# Autodesk Inventor assembly: 60-J6
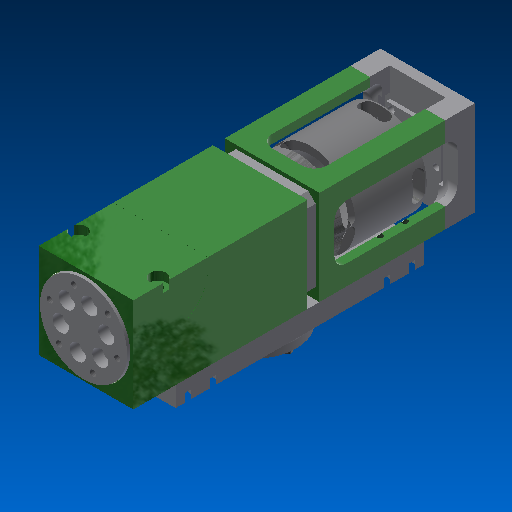
[picture p0: Inventor's stored thumbnail of the model, 512x512]
Saved by Autodesk Inventor 2018 (Build 220112000, 112)
## iProperties
Created: 2020-07-02
Part Number: 60-J6
Document SubType Name: Assembly
Designer: Bunny320
Author: Bunny320
## Documents named in this file (11)
- D:\Seerosenstr\sechs\4-CAD\60-J6.iam
- D:\Seerosenstr\sechs\4-CAD\motor unit 2820.iam
- D:\Seerosenstr\sechs\4-CAD\standardParts\61705-2RZ\W 61705-2RZ.iam
- D:\Seerosenstr\sechs\4-CAD\standardParts\Pololu mounting hub\pololu-universal-aluminum-mounting-hub-for-6mm-shaft-m3-holes.ipt
- C:\Users\Bunny320\Documents\Inventor\Content Center Files\R2018\en-US\ISO 10642(2)\ISO 10642  - M3  x  12.ipt
- C:\Users\mo\Documents\Inventor\Content Center Files\R2018\en-US\ISO 4762(1)\DIN EN ISO 4762 - M3 x 12.ipt
- C:\Users\Bunny320\Documents\Inventor\Content Center Files\R2018\en-US\ISO 4762(1)\DIN EN ISO 4762 - M3 x 8.ipt
- D:\Seerosenstr\sechs\4-CAD\602-gearbox-housing.ipt
- D:\Seerosenstr\sechs\4-CAD\601-flange.ipt
- D:\Seerosenstr\sechs\4-CAD\602-gearbox-housing-cap.ipt
- D:\Seerosenstr\sechs\4-CAD\605-output disk.ipt
## Components (25 placed, 10 different names)
1. motor unit 2820:1 [sub-assembly] — Flush:1, Flush:2, Flush:3, Mate:1, Mate:2, Mate:3, Mate:69, Mate:70
2. 602-gearbox-housing:1 — Mate:1, Mate:2, Mate:3, Mate:6, Mate:15, Mate:16, Mate:17, Mate:18, Mate:19, Mate:20, Mate:21, Mate:22, Mate:74, Mate:76, Mate:77
3. W 61705-2RZ:1 [sub-assembly] — Mate:6, Mate:71, Mate:73, Mate:74, Mate:75
4. pololu-universal-aluminum-mounting-hub-for-6mm-shaft-m3-holes:1 — Mate:72, Mate:73
5. 601-flange:1 — Mate:15, Mate:27, Mate:28, Mate:29, Mate:30, Mate:31, Mate:32, Mate:33, Mate:34, Mate:35, Mate:36, Mate:37, Mate:38, Mate:39, Mate:40, Mate:41, Mate:42, Mate:43, Mate:44, Mate:45, Mate:46, Mate:47, Mate:48, Mate:49, Mate:50, Mate:51, Mate:52, Mate:53, Mate:54, Mate:69, Mate:70
6. 602-gearbox-housing-cap:1 — Mate:16, Mate:17, Mate:18, Mate:76, Mate:77
7. 605-output disk:1 — Mate:71, Mate:72, Mate:75
8. DIN EN ISO 10642 M3  x  12:1 — Mate:19
9. DIN EN ISO 10642 M3  x  12:2 — Mate:20
10. DIN EN ISO 10642 M3  x  12:3 — Mate:21
11. DIN EN ISO 10642 M3  x  12:4 — Mate:22
12. DIN EN ISO 4762 M3 x 12:1 — Mate:27, Mate:28
13. DIN EN ISO 4762 M3 x 12:2 — Mate:29, Mate:30
14. DIN EN ISO 4762 M3 x 12:3 — Mate:31, Mate:32
15. DIN EN ISO 4762 M3 x 12:4 — Mate:33, Mate:34
16. DIN EN ISO 4762 M3 x 12:5 — Mate:35, Mate:36
17. DIN EN ISO 4762 M3 x 12:6 — Mate:37, Mate:38
18. DIN EN ISO 4762 M3 x 8:1 — Mate:39, Mate:40
19. DIN EN ISO 4762 M3 x 8:2 — Mate:41, Mate:42
20. DIN EN ISO 4762 M3 x 8:3 — Mate:43, Mate:44
21. DIN EN ISO 4762 M3 x 8:4 — Mate:45, Mate:46
22. DIN EN ISO 4762 M3 x 8:5 — Mate:47, Mate:48
23. DIN EN ISO 4762 M3 x 8:6 — Mate:49, Mate:50
24. DIN EN ISO 4762 M3 x 8:7 — Mate:51, Mate:52
25. DIN EN ISO 4762 M3 x 8:8 — Mate:53, Mate:54
## Relationships (52: Mate 49, Flush 3)
- Flush:1: motor unit 2820:1
- Flush:2: motor unit 2820:1
- Flush:3: motor unit 2820:1
- Mate:1: motor unit 2820:1 ↔ 602-gearbox-housing:1
- Mate:2: motor unit 2820:1 ↔ 602-gearbox-housing:1
- Mate:3: motor unit 2820:1 ↔ 602-gearbox-housing:1
- Mate:6: 602-gearbox-housing:1 ↔ W 61705-2RZ:1
- Mate:15: 602-gearbox-housing:1 ↔ 601-flange:1
- Mate:16: 602-gearbox-housing:1 ↔ 602-gearbox-housing-cap:1
- Mate:17: 602-gearbox-housing:1 ↔ 602-gearbox-housing-cap:1
- Mate:18: 602-gearbox-housing:1 ↔ 602-gearbox-housing-cap:1
- Mate:19: 602-gearbox-housing:1 ↔ DIN EN ISO 10642 M3  x  12:1
- Mate:20: 602-gearbox-housing:1 ↔ DIN EN ISO 10642 M3  x  12:2
- Mate:21: 602-gearbox-housing:1 ↔ DIN EN ISO 10642 M3  x  12:3
- Mate:22: 602-gearbox-housing:1 ↔ DIN EN ISO 10642 M3  x  12:4
- Mate:27: 601-flange:1 ↔ DIN EN ISO 4762 M3 x 12:1
- Mate:28: 601-flange:1 ↔ DIN EN ISO 4762 M3 x 12:1
- Mate:29: 601-flange:1 ↔ DIN EN ISO 4762 M3 x 12:2
- Mate:30: 601-flange:1 ↔ DIN EN ISO 4762 M3 x 12:2
- Mate:31: 601-flange:1 ↔ DIN EN ISO 4762 M3 x 12:3
- Mate:32: 601-flange:1 ↔ DIN EN ISO 4762 M3 x 12:3
- Mate:33: 601-flange:1 ↔ DIN EN ISO 4762 M3 x 12:4
- Mate:34: 601-flange:1 ↔ DIN EN ISO 4762 M3 x 12:4
- Mate:35: 601-flange:1 ↔ DIN EN ISO 4762 M3 x 12:5
- Mate:36: 601-flange:1 ↔ DIN EN ISO 4762 M3 x 12:5
- Mate:37: 601-flange:1 ↔ DIN EN ISO 4762 M3 x 12:6
- Mate:38: 601-flange:1 ↔ DIN EN ISO 4762 M3 x 12:6
- Mate:39: 601-flange:1 ↔ DIN EN ISO 4762 M3 x 8:1
- Mate:40: 601-flange:1 ↔ DIN EN ISO 4762 M3 x 8:1
- Mate:41: 601-flange:1 ↔ DIN EN ISO 4762 M3 x 8:2
- Mate:42: 601-flange:1 ↔ DIN EN ISO 4762 M3 x 8:2
- Mate:43: 601-flange:1 ↔ DIN EN ISO 4762 M3 x 8:3
- Mate:44: 601-flange:1 ↔ DIN EN ISO 4762 M3 x 8:3
- Mate:45: 601-flange:1 ↔ DIN EN ISO 4762 M3 x 8:4
- Mate:46: 601-flange:1 ↔ DIN EN ISO 4762 M3 x 8:4
- Mate:47: 601-flange:1 ↔ DIN EN ISO 4762 M3 x 8:5
- Mate:48: 601-flange:1 ↔ DIN EN ISO 4762 M3 x 8:5
- Mate:49: 601-flange:1 ↔ DIN EN ISO 4762 M3 x 8:6
- Mate:50: 601-flange:1 ↔ DIN EN ISO 4762 M3 x 8:6
- Mate:51: 601-flange:1 ↔ DIN EN ISO 4762 M3 x 8:7
- Mate:52: 601-flange:1 ↔ DIN EN ISO 4762 M3 x 8:7
- Mate:53: 601-flange:1 ↔ DIN EN ISO 4762 M3 x 8:8
- Mate:54: 601-flange:1 ↔ DIN EN ISO 4762 M3 x 8:8
- Mate:69: motor unit 2820:1 ↔ 601-flange:1
- Mate:70: motor unit 2820:1 ↔ 601-flange:1
- Mate:71: W 61705-2RZ:1 ↔ 605-output disk:1
- Mate:72: pololu-universal-aluminum-mounting-hub-for-6mm-shaft-m3-holes:1 ↔ 605-output disk:1
- Mate:73: W 61705-2RZ:1 ↔ pololu-universal-aluminum-mounting-hub-for-6mm-shaft-m3-holes:1
- Mate:74: 602-gearbox-housing:1 ↔ W 61705-2RZ:1
- Mate:75: W 61705-2RZ:1 ↔ 605-output disk:1
- Mate:76: 602-gearbox-housing:1 ↔ 602-gearbox-housing-cap:1
- Mate:77: 602-gearbox-housing:1 ↔ 602-gearbox-housing-cap:1
